# Autodesk Inventor assembly: TopPlate
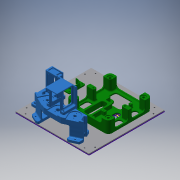
[picture p0: Inventor's stored thumbnail of the model, 180x180]
Saved by Autodesk Inventor 2016 (Build 200138000, 138)
## iProperties
Created: 2015-08-28
Part Number: TopPlate
Document SubType Name: Assembly
Designer: lachesis
Author: lachesis
## Documents named in this file (7)
- C:\Users\lachesis\Desktop\Swarmie Assembly\Assemblies\TopPlate.iam
- C:\Users\lachesis\Desktop\Swarmie Assembly\Parts\TopPlate.ipt
- C:\Users\lachesis\Desktop\Swarmie Assembly\Parts\NewGPS_IMUMount.ipt
- C:\Users\lachesis\Desktop\Swarmie Assembly\Parts\USTowerLW.ipt
- C:\Users\lachesis\Desktop\Swarmie Assembly\Parts\NewNUCBase.ipt
- C:\Users\lachesis\Desktop\Swarmie Assembly\Parts\CameraMountLW.ipt
- C:\Users\lachesis\Desktop\Swarmie Assembly\Parts\SwitchGuardLW.ipt
## Components (6 placed, 6 different names)
1. TopPlate:1 — Rigid:1, Rigid:2, Rotational:2
2. NewGPS_IMUMount:1 — Rigid:1
3. USTowerLW:1 — Rotational:1
4. NewNUCBase:1 — Rigid:2
5. CameraMountLW:1 — Rotational:1
6. SwitchGuardLW:1 — Rotational:2
## Relationships (4: WeldJoint 2, RevoluteJoint 2)
- Rigid:1 [WeldJoint]: TopPlate:1 ↔ NewGPS_IMUMount:1
- Rigid:2 [WeldJoint]: TopPlate:1 ↔ NewNUCBase:1
- Rotational:1 [RevoluteJoint]: USTowerLW:1 ↔ CameraMountLW:1
- Rotational:2 [RevoluteJoint]: TopPlate:1 ↔ SwitchGuardLW:1
